# Autodesk Inventor assembly: Greifer
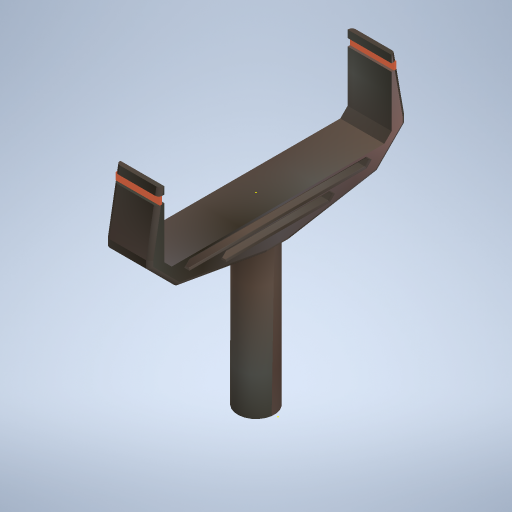
[picture p0: Inventor's stored thumbnail of the model, 512x512]
Saved by Autodesk Inventor 2023 (Build 270158000, 158)
## iProperties
Created: 2022-12-19
Part Number: Greifer
Document SubType Name: Assembly
Designer: redii
Author: redii
## Documents named in this file (3)
- C:\Users\redii\Desktop\CGM\My projectCube\Greifer.iam
- C:\Users\redii\Desktop\CGM\My projectCube\Greifer.ipt
- C:\Users\redii\Desktop\CGM\My projectCube\KontaktGreifer.ipt
## Components (3 placed, 2 different names)
1. Greifer:1 — Rigid:1, Rigid:2
2. KontaktGreifer:1 — Rigid:1
3. KontaktGreifer:2 — Rigid:2
## Relationships (2: WeldJoint 2)
- Rigid:1 [WeldJoint]: Greifer:1 ↔ KontaktGreifer:1
- Rigid:2 [WeldJoint]: Greifer:1 ↔ KontaktGreifer:2
